# Autodesk Inventor assembly: C0-1-01-ArmGearbox
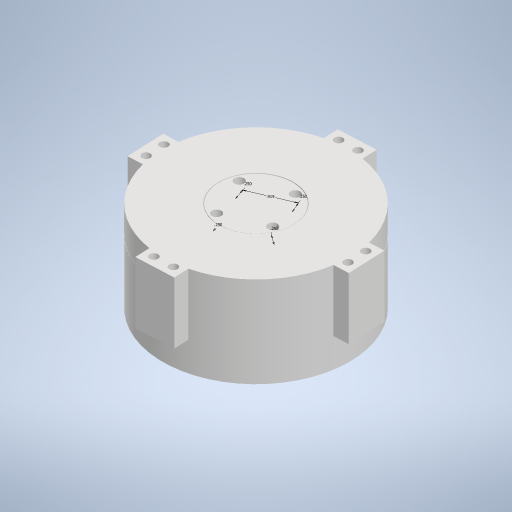
[picture p0: Inventor's stored thumbnail of the model, 512x512]
Saved by Autodesk Inventor 2023 (Build 270158000, 158)
## iProperties
Created: 2023-09-29
Part Number: C0-1-01-ArmGearbox
Document SubType Name: Assembly
Designer: thesl
Author: thesl
## Documents named in this file (5)
- C:\Users\thesl\OneDrive\Documents\GitHub\BehrendURCMechanical\CAD\Controls\C0-1-01-ArmGearbox.iam
- C:\Users\thesl\OneDrive\Documents\GitHub\BehrendURCMechanical\CAD\Controls\CO-0-01-ArmMotorMount.ipt
- C:\Users\thesl\OneDrive\Documents\GitHub\BehrendURCMechanical\CAD\Controls\CO-1-01-armMotor.ipt
- C:\Users\thesl\OneDrive\Documents\GitHub\BehrendURCMechanical\CAD\Controls\CO-0-01-Planetary1.ipt
- C:\Users\thesl\OneDrive\Documents\GitHub\BehrendURCMechanical\CAD\Controls\CO-0-01-PlanetaryCap.ipt
## Components (4 placed, 4 different names)
1. CO-0-01-ArmMotorMount:1 — Insert:2, Insert:3, Insert:4, Insert:7, Insert:8
2. CO-1-01-armMotor:1 — Insert:2, Insert:3, Insert:4, Insert:5, Insert:6
3. CO-0-01-Planetary1:1 — Insert:5, Insert:6
4. CO-0-01-PlanetaryCap:1 — Insert:7, Insert:8
## Relationships (7: Insert 7)
- Insert:2 (-6.35 mm): CO-0-01-ArmMotorMount:1 ↔ CO-1-01-armMotor:1
- Insert:3 (6.35 mm): CO-0-01-ArmMotorMount:1 ↔ CO-1-01-armMotor:1
- Insert:4 (6.35 mm): CO-0-01-ArmMotorMount:1 ↔ CO-1-01-armMotor:1
- Insert:5: CO-1-01-armMotor:1 ↔ CO-0-01-Planetary1:1
- Insert:6: CO-1-01-armMotor:1 ↔ CO-0-01-Planetary1:1
- Insert:7: CO-0-01-ArmMotorMount:1 ↔ CO-0-01-PlanetaryCap:1
- Insert:8: CO-0-01-ArmMotorMount:1 ↔ CO-0-01-PlanetaryCap:1
